# Autodesk Inventor assembly: Assembly1
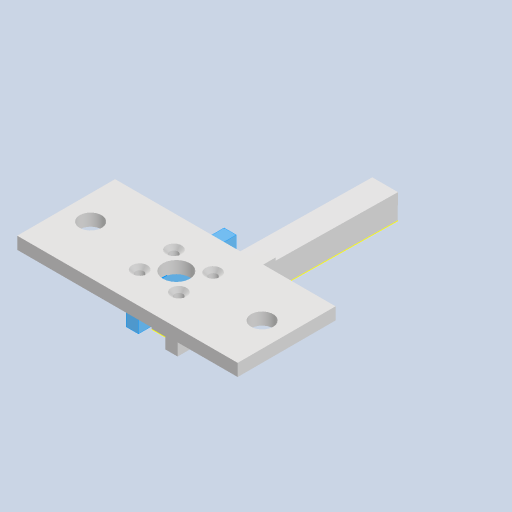
[picture p0: Inventor's stored thumbnail of the model, 512x512]
Saved by Autodesk Inventor 2023.4 (Build 274418000, 418)
## iProperties
Created: 2024-01-12
Part Number: Assembly1
Document SubType Name: Assembly
Designer: PalumaCMM
Author: PalumaCMM
## Documents named in this file (4)
- C:\Users\PalumaCMM\Documents\Inventor\Sucharitha\Safety mechanism\Assembly1.iam
- C:\Users\PalumaCMM\Documents\Inventor\Sucharitha\Al Attach block.ipt
- C:\Users\PalumaCMM\Documents\Inventor\Sucharitha\Al block2.ipt
- C:\Users\PalumaCMM\Documents\Inventor\Sucharitha\Flange.ipt
## Components (4 placed, 3 different names)
1. Al block2:1 — Mate:8, Mate:9, Mate:10, Mate:11, Mate:12, Mate:13, Mate:14, Mate:15, Mate:16
2. Al Attach block:1 — Mate:11, Mate:12, Mate:13, Mate:17
3. Al Attach block:2 — Mate:14, Mate:15, Mate:16, Mate:18
4. Flange:1 — Mate:17, Mate:18
## Relationships (11: Mate 11)
- Mate:8: Al block2:1
- Mate:9: Al block2:1
- Mate:10: Al block2:1
- Mate:11: Al block2:1 ↔ Al Attach block:1
- Mate:12: Al block2:1 ↔ Al Attach block:1
- Mate:13: Al block2:1 ↔ Al Attach block:1
- Mate:14: Al block2:1 ↔ Al Attach block:2
- Mate:15: Al block2:1 ↔ Al Attach block:2
- Mate:16: Al block2:1 ↔ Al Attach block:2
- Mate:17: Al Attach block:1 ↔ Flange:1
- Mate:18: Al Attach block:2 ↔ Flange:1
